# Autodesk Inventor assembly: Build
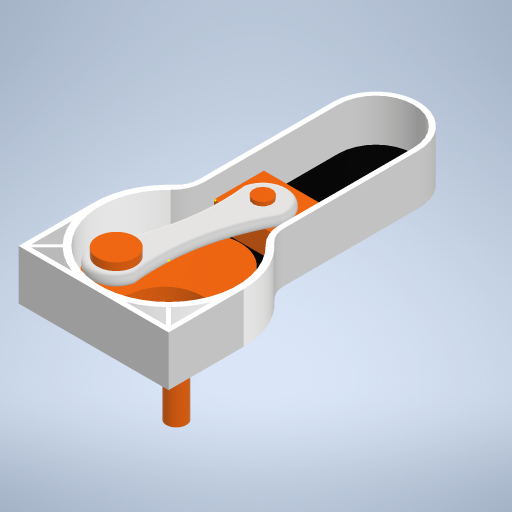
[picture p0: Inventor's stored thumbnail of the model, 512x512]
Saved by Autodesk Inventor 2024 (Build 280153020, 153B)
## iProperties
Created: 2023-09-12
Part Number: Build
Document SubType Name: Assembly
Designer: 23also
Author: 23also
## Documents named in this file (8)
- C:\Users\23also\Inventor\Combustion Engine\Build.iam
- C:\Users\23also\Inventor\Combustion Engine\Axel chamber.ipt
- C:\Users\23also\Inventor\Combustion Engine\Axel.ipt
- C:\Users\23also\Inventor\Combustion Engine\Arm.ipt
- C:\Users\23also\Inventor\Combustion Engine\Kolv.ipt
- C:\Users\23also\Inventor\Combustion Engine\Kolv knapp.ipt
- C:\Users\23also\Inventor\Combustion Engine\Axel knapp.ipt
- C:\Users\23also\Inventor\Combustion Engine\Vevarm.ipt
## Components (7 placed, 7 different names)
1. Axel chamber:1 — Mate:4, Rotational:1, Mate:9
2. Axel:1 — Cylindrical:7, Mate:6, Rigid:1
3. Arm:1 — Cylindrical:5, Cylindrical:6, Mate:5, Mate:8
4. Kolv:1 — Mate:4, Cylindrical:4, Mate:7, Mate:9
5. Kolv knapp:1 — Cylindrical:4, Cylindrical:5, Mate:7, Mate:8
6. Axel knapp:1 — Cylindrical:6, Cylindrical:7, Mate:5, Mate:6
7. Vevarm:1 — Rigid:1, Rotational:1
## Relationships (12: Mate 6, CylindricalJoint 4, WeldJoint 1, RevoluteJoint 1)
- Mate:4 (1 mm): Axel chamber:1 ↔ Kolv:1
- Cylindrical:4: Kolv:1 ↔ Kolv knapp:1
- Cylindrical:5: Arm:1 ↔ Kolv knapp:1
- Cylindrical:6: Arm:1 ↔ Axel knapp:1
- Cylindrical:7: Axel:1 ↔ Axel knapp:1
- Mate:5 (0.5 mm): Arm:1 ↔ Axel knapp:1
- Mate:6: Axel:1 ↔ Axel knapp:1
- Mate:7: Kolv:1 ↔ Kolv knapp:1
- Rigid:1 [WeldJoint]: Axel:1 ↔ Vevarm:1
- Rotational:1 [RevoluteJoint]: Axel chamber:1 ↔ Vevarm:1
- Mate:8 (0.5 mm): Arm:1 ↔ Kolv knapp:1
- Mate:9 (0.5 mm): Axel chamber:1 ↔ Kolv:1
